# Autodesk Inventor assembly: 775pro_1_Female
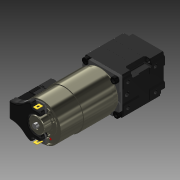
[picture p0: Inventor's stored thumbnail of the model, 180x180]
Saved by Autodesk Inventor 2022 (Build 260153000, 153)
## iProperties
Created: 2018-08-19
Part Number: 775pro_1_Female
Document SubType Name: Assembly
Mass: 1123.04 g
Surface Area: 1203.25 cm^2
Volume: 285.054 cm^3
Density: 3.93975 g/cm^3
## Documents named in this file (10)
- C:\Users\Cal\Desktop\Robotics\Design\Collaborative\Collaborative Parts Library\General Gearboxes\Planetaries\Versaplanetary\VersaPlanetary\775pro, 1 Stages, Female Output.iam
- C:\Users\Cal\Desktop\Robotics\Design\Collaborative\Collaborative Parts Library\General Gearboxes\Planetaries\Versaplanetary\V2 Stages\V2 Output Stage.iam
- C:\Users\Cal\Desktop\Robotics\Design\Collaborative\Collaborative Parts Library\General Gearboxes\Planetaries\Versaplanetary\Intermediate Stages\Ring Gear.ipt
- C:\Users\Cal\Desktop\Robotics\Design\Collaborative\Collaborative Parts Library\General Gearboxes\Planetaries\Versaplanetary\V2 Stages\V2 Input Stage.iam
- C:\Users\Cal\Desktop\Robotics\Design\Collaborative\Collaborative Parts Library\General Gearboxes\Planetaries\Versaplanetary\Screws\8-32 x 1.75in Screw.ipt
- C:\Users\Cal\Desktop\Robotics\Design\Collaborative\Collaborative Parts Library\Power Transfer\Bearings and Bushings\Bearings\6902ZZ.ipt
- E:\Middleton Robotics\Collaborative Robots\Collaborative Part Library\Power Transfer\Bearings.ipt
- C:\Users\Cal\Desktop\Robotics\Design\Collaborative\Collaborative Parts Library\General Gearboxes\Planetaries\Versaplanetary\V2 Stages\V2 Input Stage\VP 775pro Input.iam
- C:\Users\Cal\Desktop\Robotics\Design\Collaborative\Collaborative Parts Library\General Gearboxes\Planetaries\Versaplanetary\VersaPlanetary.iam
- C:\Users\Cal\Desktop\Robotics\Design\Collaborative\Collaborative Parts Library\General Gearboxes\Planetaries\Versaplanetary\V2 Stages\V2 Output Stage\VP V2 Output Stage Female.iam
## Components (7 placed, 5 different names)
1. VP V2 Output Stage Female:3 [sub-assembly] — Insert:1, Flush:3, Insert:25
2. Ring Gear 1 — Insert:1, Flush:3, 1StageBasicInputMate1, 1StageBasicInputMate2
3. VP 775pro Input:1 [sub-assembly] — 1StageBasicInputMate1, 1StageBasicInputMate2, Insert:8, Insert:9
4. 8-32 x 1.75in Screw:1 — Insert:8
5. 8-32 x 1.75in Screw:2 — Insert:9
6. 6902ZZ:1
7. 6902ZZ:2 — Insert:25
## Relationships (7: Insert 5, Flush 2)
- Insert:1: VP V2 Output Stage Female:3 ↔ Ring Gear 1
- Flush:3: VP V2 Output Stage Female:3 ↔ Ring Gear 1
- 1StageBasicInputMate1 [Insert]: Ring Gear 1 ↔ VP 775pro Input:1
- 1StageBasicInputMate2 [Flush]: Ring Gear 1 ↔ VP 775pro Input:1
- Insert:8: VP 775pro Input:1 ↔ 8-32 x 1.75in Screw:1
- Insert:9: VP 775pro Input:1 ↔ 8-32 x 1.75in Screw:2
- Insert:25: VP V2 Output Stage Female:3 ↔ 6902ZZ:2
